# Autodesk Inventor assembly: OringFixture
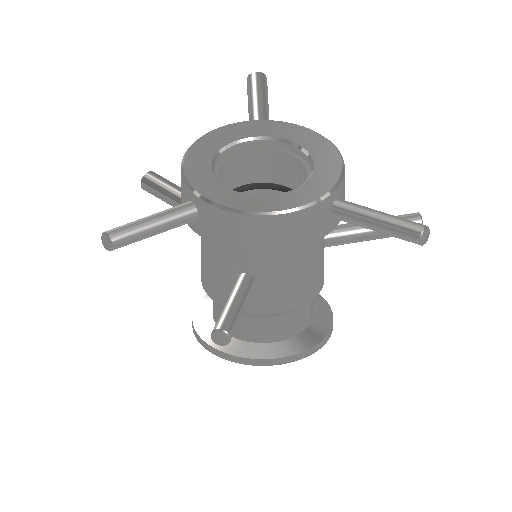
[picture p0: Inventor's stored thumbnail of the model, 512x512]
Saved by Autodesk Inventor 2026.2 (Build 302298000, 298)
## iProperties
Created: 2022-12-02
Part Number: OringFixture
Document SubType Name: Assembly
Designer: kuzmin
Author: kuzmin
## Documents named in this file (6)
- D:\repos\PIHTI\Plasma Vessel_2026\contents\OringFixture.iam
- D:\repos\PIHTI\PALP\Oring-seal\Oring_KF_part.iam
- D:\repos\PIHTI\PALP\Oring-seal\OringPressingRing.ipt
- D:\repos\PIHTI\PALP\Oring-seal\Oring.ipt
- D:\repos\PIHTI\PALP\Oring-seal\Oring_M48-2_nut.ipt
- D:\repos\PIHTI\PALP\Oring-seal\OringM5Wrench.ipt
## Components (10 placed, 5 different names)
1. Oring_KF_part:1 [sub-assembly] — メイト:1, メイト:2, メイト:3, メイト:4, 正接:1, メイト:5, リジッド:1, リジッド:2, リジッド:3
2. OringPressingRing:1 — メイト:5, 正接:2, 回転:1
3. Oring:1 — メイト:4, 正接:1, 正接:2
4. Oring_M48-2_nut:1 — 回転:1, 回転:2, 回転:3, 回転:4
5. OringM5Wrench:1 — 回転:2
6. OringM5Wrench:2 — 回転:4
7. OringM5Wrench:3 — 回転:3
8. OringM5Wrench:4 — リジッド:1
9. OringM5Wrench:5 — リジッド:2
10. OringM5Wrench:6 — リジッド:3
## Relationships (14: Mate 5, RevoluteJoint 4, WeldJoint 3, Tangent 2)
- メイト:1 [Mate]: Oring_KF_part:1
- メイト:2 [Mate]: Oring_KF_part:1
- メイト:3 [Mate]: Oring_KF_part:1
- メイト:4 [Mate]: Oring_KF_part:1 ↔ Oring:1
- 正接:1 [Tangent]: Oring_KF_part:1 ↔ Oring:1
- メイト:5 [Mate]: Oring_KF_part:1 ↔ OringPressingRing:1
- 正接:2 [Tangent]: OringPressingRing:1 ↔ Oring:1
- 回転:1 [RevoluteJoint]: OringPressingRing:1 ↔ Oring_M48-2_nut:1
- 回転:2 [RevoluteJoint]: Oring_M48-2_nut:1 ↔ OringM5Wrench:1
- 回転:3 [RevoluteJoint]: Oring_M48-2_nut:1 ↔ OringM5Wrench:3
- 回転:4 [RevoluteJoint]: Oring_M48-2_nut:1 ↔ OringM5Wrench:2
- リジッド:1 [WeldJoint]: Oring_KF_part:1 ↔ OringM5Wrench:4
- リジッド:2 [WeldJoint]: Oring_KF_part:1 ↔ OringM5Wrench:5
- リジッド:3 [WeldJoint]: Oring_KF_part:1 ↔ OringM5Wrench:6
